# Autodesk Inventor assembly: BearingWithInsert
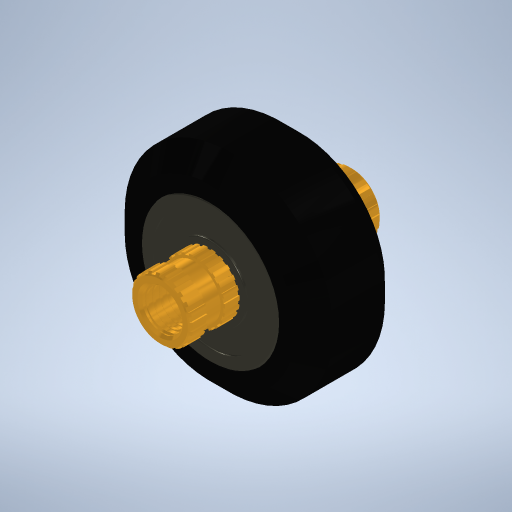
[picture p0: Inventor's stored thumbnail of the model, 512x512]
Saved by Autodesk Inventor 2024.2 (Build 282272000, 272)
## iProperties
Created: 2025-04-11
Part Number: BearingWithInsert
Document SubType Name: Assembly
Designer: Admin
Author: Admin
## Documents named in this file (3)
- C:\Users\Admin\Documents\GitHub\GripperPropuesto\Assemblies\BearingWithInsert.iam
- C:\Users\Admin\Documents\GitHub\GripperPropuesto\AuxiliarPieces\M5x6-Insert\M5x6-Insert.ipt
- C:\Users\Admin\Documents\GitHub\GripperPropuesto\AuxiliarPieces\NylonBearing\NylonPulleyBearing.iam
## Components (3 placed, 2 different names)
1. M5x6-Insert:1 — Mate:1, Mate:2
2. NylonPulleyBearing:1 [sub-assembly] — Mate:1, Mate:2, Mate:3, Mate:4
3. M5x6-Insert:2 — Mate:3, Mate:4
## Relationships (4: Mate 4)
- Mate:1: M5x6-Insert:1 ↔ NylonPulleyBearing:1
- Mate:2: M5x6-Insert:1 ↔ NylonPulleyBearing:1
- Mate:3: NylonPulleyBearing:1 ↔ M5x6-Insert:2
- Mate:4: NylonPulleyBearing:1 ↔ M5x6-Insert:2
